# Autodesk Inventor assembly: złożenie nr1
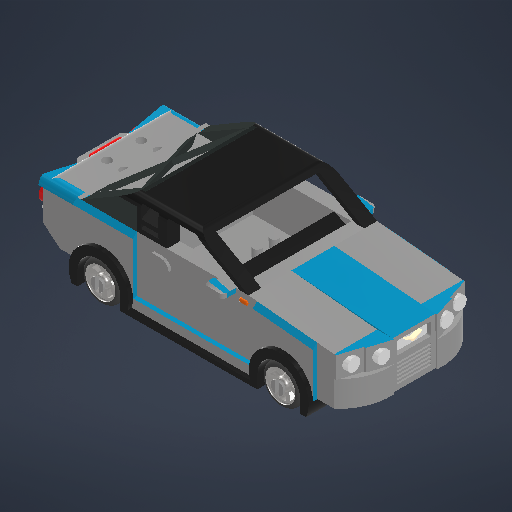
[picture p0: Inventor's stored thumbnail of the model, 512x512]
Saved by Autodesk Inventor 2026.2 (Build 302298000, 298)
## iProperties
Created: 2026-08-16
Part Number: złożenie nr1
Document SubType Name: Assembly
Designer: wojsl
Author: wojsl
## Documents named in this file (5)
- C:\Users\wojsl\OneDrive\Pulpit\cad\samochód\złożenie nr1.iam
- C:\Users\wojsl\OneDrive\Pulpit\cad\samochód\main.ipt
- C:\Users\wojsl\OneDrive\Pulpit\cad\samochód\opona.ipt
- C:\Users\wojsl\OneDrive\Pulpit\cad\samochód\zderzak.ipt
- C:\Users\wojsl\OneDrive\Pulpit\cad\samochód\dach.ipt
## Components (7 placed, 4 different names)
1. main:1 — Wstawiające:1, Wstawiające:2, Wstawiające:3, Wstawiające:4, Wstawiające:5, Wstawiające:6, Wstawiające:7, Wstawiające:8
2. opona:1 — Wstawiające:4
3. opona:2 — Wstawiające:3
4. opona:3 — Wstawiające:2
5. opona:4 — Wstawiające:1
6. zderzak:1 — Wstawiające:5, Wstawiające:6
7. dach:1 — Wstawiające:7, Wstawiające:8
## Relationships (8: Insert 8)
- Wstawiające:1 [Insert]: main:1 ↔ opona:4
- Wstawiające:2 [Insert]: main:1 ↔ opona:3
- Wstawiające:3 [Insert]: main:1 ↔ opona:2
- Wstawiające:4 [Insert]: main:1 ↔ opona:1
- Wstawiające:5 [Insert]: main:1 ↔ zderzak:1
- Wstawiające:6 [Insert]: main:1 ↔ zderzak:1
- Wstawiające:7 [Insert]: main:1 ↔ dach:1
- Wstawiające:8 [Insert]: main:1 ↔ dach:1
